# Autodesk Inventor assembly: Liu_Inital_Assably
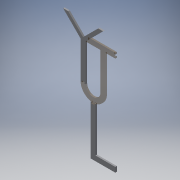
[picture p0: Inventor's stored thumbnail of the model, 180x180]
Saved by Autodesk Inventor 2017 (Build 210142000, 142)
## iProperties
Created: 2016-09-23
Part Number: Liu_Inital_Assably
Document SubType Name: Assembly
Designer: jliu
Author: jliu
## Documents named in this file (4)
- R:\Engineering\Eng16-17\CAD-CAM\Jinyu Liu\Project 2 Initals\Initals\Liu_Inital_Assably.iam
- R:\Engineering\Eng16-17\CAD-CAM\Jinyu Liu\Project 2 Initals\Initals\Liu_Inital_J.ipt
- R:\Engineering\Eng16-17\CAD-CAM\Jinyu Liu\Project 2 Initals\Initals\Liu_Inital_Y.ipt
- R:\Engineering\Eng16-17\CAD-CAM\Jinyu Liu\Project 2 Initals\Initals\Liu_Inital_L.ipt
## Components (3 placed, 3 different names)
1. Liu_Inital_J:1 — Mate:1, Flush:1, Mate:2, Mate:3, Mate:4, Flush:2
2. Liu_Inital_Y:1 — Mate:1, Flush:1, Mate:2
3. Liu_Inital_L:1 — Mate:3, Mate:4, Flush:2
## Relationships (6: Mate 4, Flush 2)
- Mate:1: Liu_Inital_J:1 ↔ Liu_Inital_Y:1
- Flush:1: Liu_Inital_J:1 ↔ Liu_Inital_Y:1
- Mate:2: Liu_Inital_J:1 ↔ Liu_Inital_Y:1
- Mate:3: Liu_Inital_J:1 ↔ Liu_Inital_L:1
- Mate:4: Liu_Inital_J:1 ↔ Liu_Inital_L:1
- Flush:2: Liu_Inital_J:1 ↔ Liu_Inital_L:1
